# Autodesk Inventor assembly: McCrea_RUKA_Walle_MIR
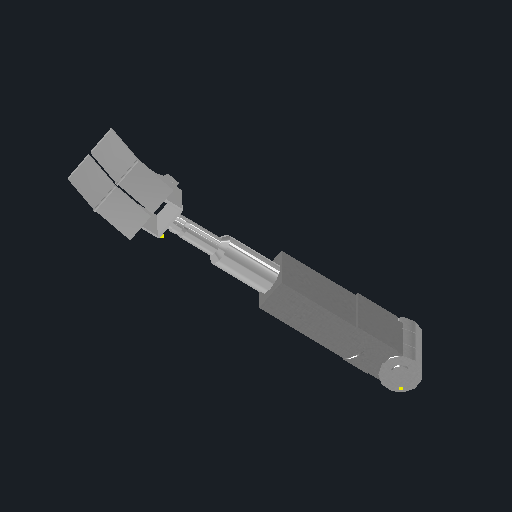
[picture p0: Inventor's stored thumbnail of the model, 512x512]
Saved by Autodesk Inventor 2022 (Build 260153000, 153)
## iProperties
Created: 2022-01-25
Part Number: McCrea_RUKA_Walle_MIR
Document SubType Name: Assembly
Designer: MatusBarany
Author: Lukas
## Documents named in this file (7)
- C:\Users\MatusBarany\Documents\Inventor\wall-e\lukas\McCrea_RUKA_Walle_MIR.iam
- C:\Users\MatusBarany\Documents\Inventor\wall-e\lukas\McCrea_rameno_Walle_MIR.ipt
- C:\Users\MatusBarany\Documents\Inventor\wall-e\lukas\McCrea_paza_Walle_MIR.ipt
- C:\Users\MatusBarany\Documents\Inventor\wall-e\lukas\McCrea_wrist_Walle_MIR.ipt
- C:\Users\MatusBarany\Documents\Inventor\wall-e\lukas\McCrea_arm-connector_Walle_MIR.ipt
- C:\Users\MatusBarany\Documents\Inventor\wall-e\lukas\McCrea_finger_Walle_MIR.ipt
- C:\Users\MatusBarany\Documents\Inventor\wall-e\lukas\McCrea_finger2_Walle_MIR.ipt
## Components (6 placed, 6 different names)
1. McCrea_rameno_Walle_MIR:1 — Flush:1, Cylindrical:1
2. McCrea_paza_Walle_MIR:1 — Flush:1, Cylindrical:1, Rigid:1
3. McCrea_wrist_Walle_MIR:1 — Rigid:1, Rotational:1
4. McCrea_arm-connector_Walle_MIR:1 — Rotational:1, Rotational:2, Rotational:3
5. McCrea_finger_Walle_MIR:1 — Rotational:2
6. McCrea_finger2_Walle_MIR:1 — Rotational:3
## Relationships (6: RevoluteJoint 3, Flush 1, CylindricalJoint 1, WeldJoint 1)
- Flush:1: McCrea_rameno_Walle_MIR:1 ↔ McCrea_paza_Walle_MIR:1
- Cylindrical:1: McCrea_rameno_Walle_MIR:1 ↔ McCrea_paza_Walle_MIR:1
- Rigid:1 [WeldJoint]: McCrea_paza_Walle_MIR:1 ↔ McCrea_wrist_Walle_MIR:1
- Rotational:1 [RevoluteJoint]: McCrea_wrist_Walle_MIR:1 ↔ McCrea_arm-connector_Walle_MIR:1
- Rotational:2 [RevoluteJoint]: McCrea_arm-connector_Walle_MIR:1 ↔ McCrea_finger_Walle_MIR:1
- Rotational:3 [RevoluteJoint]: McCrea_arm-connector_Walle_MIR:1 ↔ McCrea_finger2_Walle_MIR:1
